# Autodesk Inventor assembly: Baugruppe2
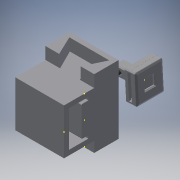
[picture p0: Inventor's stored thumbnail of the model, 180x180]
Saved by Autodesk Inventor 2017 (Build 210142000, 142)
## iProperties
Part Number: Baugruppe2
Material: Generisch
Document SubType Name: Assembly
Designer: Skenderbeg
Author: Skenderbeg
## Documents named in this file (7)
- C:\Users\Skenderbeg\Desktop\Seminar Abschluss\Raspberrycamhalter\Baugruppe2.iam
- C:\Users\Skenderbeg\Desktop\Seminar 2018\21052018 Stick\Freiburg seminar\Schwalbenschwanz Gegenstück für Cam.ipt
- C:\Users\Skenderbeg\Desktop\Seminar 2018\21052018 Stick\Freiburg seminar\Schienenaufsatz mitKeil.ipt
- C:\Users\Skenderbeg\Documents\Inventor\Content Center Files\R2017\de-DE\ISO 4036(2)\ISO 4036 - M4(2).ipt
- C:\Users\Skenderbeg\Documents\Inventor\Content Center Files\R2017\de-DE\ISO 7046-1 Z(1)\ISO 7046-1 - M4 x 40 - 4.8 - Z - ISO.ipt
- C:\Users\Skenderbeg\Desktop\Seminar 2018\21052018 Stick\Bauteil6.ipt
- C:\Users\Skenderbeg\Desktop\Seminar 2018\21052018 Stick\Bauteil7.ipt
## Components (6 placed, 6 different names)
1. Schwalbenschwanz Gegenstück für Cam:1 — Verschiebbar:1, Einfügen:1
2. Schienenaufsatz mitKeil:1 — Verschiebbar:1
3. ISO 4036 M4:1 — Einfügen:2
4. ISO 7046-1 Z M4 x 40 - 4.8 - Z:1 — Einfügen:1, Einfügen:2, Einfügen:3
5. Bauteil6:1 — Starr:1
6. Bauteil7:1 — Starr:1, Einfügen:3
## Relationships (5: Insert 3, TranslationJoint 1, WeldJoint 1)
- Verschiebbar:1 [TranslationJoint]: Schwalbenschwanz Gegenstück für Cam:1 ↔ Schienenaufsatz mitKeil:1
- Einfügen:1 [Insert]: Schwalbenschwanz Gegenstück für Cam:1 ↔ ISO 7046-1 Z M4 x 40 - 4.8 - Z:1
- Einfügen:2 [Insert] (32 mm): ISO 4036 M4:1 ↔ ISO 7046-1 Z M4 x 40 - 4.8 - Z:1
- Starr:1 [WeldJoint]: Bauteil6:1 ↔ Bauteil7:1
- Einfügen:3 [Insert]: ISO 7046-1 Z M4 x 40 - 4.8 - Z:1 ↔ Bauteil7:1
